# Autodesk Inventor assembly: Arm 2.0 Assembly
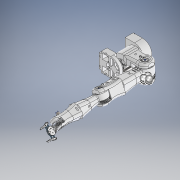
[picture p0: Inventor's stored thumbnail of the model, 180x180]
Saved by Autodesk Inventor 2017 SP1 (Build 210196100, 196)
## iProperties
Created: 2017-09-28
Part Number: Arm 2.0 Assembly
Document SubType Name: Assembly
Designer: Zach
Author: Zach
## Documents named in this file (49)
- C:\Users\Zach\Documents\GitHub\tr1\src\Body\Arm 2.0 Assembly\Arm 2.0 Assembly.iam
- C:\Users\Zach\Documents\GitHub\tr1\src\Body\Arm 2.0 Assembly\Steel Rod 8mm x 135mm.ipt
- C:\Users\Zach\Documents\GitHub\tr1\lib\22x8x8mm Bearing.ipt
- C:\Users\Zach\Documents\GitHub\tr1\src\Body\Arm 2.0 Assembly\AA004.ipt
- C:\Users\Zach\Documents\GitHub\tr1\lib\QS12MM250\QS12MM250.ipt
- C:\Users\Zach\Documents\GitHub\tr1\src\Body\Arm 2.0 Assembly\Steel Rod 8mm x 100mm.ipt
- C:\Users\Zach\Documents\GitHub\tr1\src\Body\Arm 2.0 Assembly\AA013.ipt
- C:\Users\Zach\Documents\GitHub\tr1\src\Body\Arm 2.0 Assembly\AA014.ipt
- C:\Users\Zach\Documents\GitHub\tr1\lib\12V DC Motor 378-1.ipt
- C:\Users\Zach\Documents\Inventor\Content Center Files\R2017\en-US\ISO 4017(1)\ISO 4017 - M5 x 20 - ISO.ipt
- C:\Users\Zach\Documents\GitHub\tr1\src\Body\Arm 2.0 Assembly\Steel Rod 8mm x 80mm.ipt
- C:\Users\Zach\Documents\GitHub\BCN3D-Moveo\Autodesk Inventor files\Gripper B Assembly.iam
- C:\Users\Zach\Documents\Inventor\Content Center Files\R2017\en-US\CNS 4320\CNS 4320 - M8 x 1 x 100.ipt
- C:\Users\Zach\Documents\GitHub\tr1\lib\AS 1110 - M8 x 150.ipt
- C:\Users\Zach\Documents\GitHub\tr1\lib\8mm Hub.ipt
- C:\Users\Zach\Documents\GitHub\tr1\src\Body\Arm 2.0 Assembly\Arm 2.0 Assembly\Design Accelerator\Spur Gears5.iam
- C:\Users\Zach\Documents\GitHub\tr1\lib\4mm mounting hub.ipt
- C:\Users\Zach\Documents\GitHub\tr1\lib\6201RS\6201RS.ipt
- C:\Users\Zach\Documents\GitHub\tr1\lib\U51105\U51105.ipt
- C:\Users\Zach\Documents\GitHub\tr1\src\Body\Arm 2.0 Assembly\AA031.ipt
- C:\Users\Zach\Documents\GitHub\tr1\src\Body\Arm 2.0 Assembly\AA034.ipt
- C:\Users\Zach\Documents\GitHub\tr1\src\Body\Arm 2.0 Assembly\Arm 2.0 Assembly\Design Accelerator\Spur Gears6.iam
- C:\Users\Zach\Documents\GitHub\tr1\src\Body\Arm 2.0 Assembly\AA008c.ipt
- C:\Users\Zach\Documents\GitHub\tr1\src\Body\Arm 2.0 Assembly\AA008d.ipt
- C:\Users\Zach\Documents\GitHub\tr1\src\Body\Arm 2.0 Assembly\AA035.ipt
- C:\Users\Zach\Documents\GitHub\tr1\src\Body\Arm 2.0 Assembly\Arm 2.0 Assembly\Design Accelerator\Spur Gears7.iam
- C:\Users\Zach\Documents\GitHub\tr1\src\Body\Arm 2.0 Assembly\AA036.ipt
- C:\Users\Zach\Documents\GitHub\tr1\src\Body\Arm 2.0 Assembly\AA037.ipt
- C:\Users\Zach\Documents\GitHub\tr1\src\Body\Arm 2.0 Assembly\AA016b.ipt
- C:\Users\Zach\Documents\GitHub\tr1\src\Body\Arm 2.0 Assembly\AA005b.ipt
- C:\Users\Zach\Documents\GitHub\tr1\src\Body\Arm 2.0 Assembly\AA006b.ipt
- C:\Users\Zach\Documents\GitHub\tr1\src\Body\Arm 2.0 Assembly\AA001c.ipt
- C:\Users\Zach\Documents\GitHub\tr1\lib\uxcell 12V 5RPM 8mm Worm Gear Motor\uxcell 12V 5RPM 8mm Worm Gear Motor.ipt
- C:\Users\Zach\Documents\GitHub\tr1\lib\Bourns ACE 128\Bourns ACE 128.ipt
- C:\Users\Zach\Documents\GitHub\tr1\src\Body\Arm 2.0 Assembly\Arm 2.0 Assembly\Design Accelerator\Spur Gears8.iam
- C:\Users\Zach\Documents\GitHub\tr1\src\Body\Arm 2.0 Assembly\Arm 2.0 Assembly\Design Accelerator\Spur Gears11.iam
- C:\Users\Zach\Documents\GitHub\tr1\src\Body\Arm 2.0 Assembly\Arm 2.0 Assembly\Design Accelerator\Spur Gears9.iam
- C:\Users\Zach\Documents\GitHub\tr1\src\Body\Arm 2.0 Assembly\AA010b.ipt
- C:\Users\Zach\Documents\GitHub\tr1\lib\uxcell 12V 6RPM 6mm Worm Gear Motor\uxcell 12V 6RPM 6mm Worm Gear Motor.ipt
- C:\Users\Zach\Documents\GitHub\tr1\src\Body\Arm 2.0 Assembly\Arm 2.0 Assembly\Design Accelerator\Spur Gears10.iam
- C:\Users\Zach\Documents\GitHub\tr1\src\Body\Arm 2.0 Assembly\Arm 2.0 Assembly\Design Accelerator\Spur Gears12.iam
- C:\Users\Zach\Documents\GitHub\tr1\src\Body\Arm 2.0 Assembly\AA041.ipt
- C:\Users\Zach\Documents\GitHub\tr1\src\Body\Arm 2.0 Assembly\AA042.ipt
- C:\Users\Zach\Documents\Inventor\Content Center Files\R2017\en-US\ISO 7045  H\ISO 7045 - M3 x 8 - 4.8 - H - ISO.ipt
- C:\Users\Zach\Documents\GitHub\tr1\src\Body\Arm 2.0 Assembly\AA043.ipt
- C:\Users\Zach\Documents\GitHub\tr1\src\Body\Arm 2.0 Assembly\AA044.ipt
- C:\Users\Zach\Documents\GitHub\tr1\src\Body\Arm 2.0 Assembly\AA045.ipt
- C:\Users\Zach\Documents\GitHub\tr1\src\Body\Arm 2.0 Assembly\Arm 2.0 Assembly\Design Accelerator\Spur Gears13.iam
- C:\Users\Zach\Documents\GitHub\tr1\src\Body\Arm 2.0 Assembly\Arm 2.0 Assembly\Design Accelerator\Spur Gears16.iam
## Components (84 placed, 39 different names)
1. AA001c:1 — Mate:554, Mate:555, Mate:556, Mate:557, Mate:560, Flush:18, Mate:562, Mate:563, Mate:564, Mate:565, Mate:566, Mate:567, Mate:568, Mate:569, Mate:570, Mate:571, Mate:572, Mate:573, Mate:574, Mate:576, Mate:578, Mate:581, Angle:1, Mate:592, Mate:602
2. AA004:1 — Mate:23, Mate:345, Mate:347, Mate:350, Mate:357, Mate:554, Mate:555, Mate:556, Mate:590, Mate:591
3. AA005b:1 — Mate:537, Mate:538, Mate:539, Mate:541, Mate:542, Mate:543
4. AA006b:1 — Mate:544, Mate:583, Mate:584, Angle:2, Mate:588, Mate:593, Mate:594, Mate:598, Mate:599, Mate:600, Mate:609
5. AA008c:1 — Mate:449, Mate:450, Mate:451, Mate:452, Mate:453, Mate:454, Mate:463, Mate:464, Mate:466, Mate:467, Mate:481, Mate:616, Mate:662, Mate:663
6. AA008d:1 — Mate:455, Mate:456, Mate:457, Mate:461, Mate:463, Mate:464, Mate:466, Mate:467, Mate:614, Angle:4, Mate:635, Mate:662, Mate:663, Mate:697, Mate:699
7. AA010b:1 — Mate:615, Mate:616, Mate:617, Mate:618, Mate:620, Mate:621, Mate:623, Mate:624, Mate:625, Mate:626, Mate:628, Mate:630, Mate:632, Mate:633, Mate:634, Mate:636, Mate:637, Angle:6, Mate:642, Flush:20, Mate:648, Mate:650
8. AA013:2 — Mate:142, Mate:143, Mate:144, Mate:145, Mate:146, Mate:147, Mate:563, Mate:564, Mate:565
9. AA014:2 — Mate:628, Mate:629, Mate:630
10. AA016b:1 — Mate:518, Mate:519, Mate:520, Mate:521, Mate:525, Mate:526, Mate:527, Mate:529, Mate:530, Mate:664, Mate:665, Mate:667, Mate:668, Mate:669, Angle:7, Mate:671, Mate:673, Mate:675, Mate:676, Mate:677
11. AA031:1 — Mate:366, Mate:367, Mate:523, Mate:524
12. AA034:1 — Mate:529, Mate:534, Mate:535, Mate:700, Mate:701, Mate:709
13. AA035:1 — Mate:477, Mate:479, Mate:481, Mate:557, Mate:601, Mate:652, Mate:653, Mate:697, Mate:699
14. AA036:1 — Mate:498, Mate:500, Mate:501, Mate:502, Mate:511, Mate:698
15. AA037:1 — Mate:501, Mate:502, Mate:514, Mate:515, Mate:516, Mate:517, Mate:518, Mate:519, Mate:520, Mate:530, Mate:664, Mate:665, Mate:698
16. AA041:1 — Mate:675, Mate:676, Mate:677, Mate:682, Mate:683, Mate:684, Mate:685
17. AA042:1 — Mate:678, Mate:679, Mate:686, Mate:687
18. AA043:1 — Mate:688, Mate:689, Angle:8
19. AA043:2 — Mate:693, Mate:694, Angle:10
20. AA044:1 — Mate:691, Mate:692, Angle:9
21. AA044:2 — Mate:695, Mate:696, Angle:11
22. AA045:2 — Mate:700, Mate:701, Mate:702, Mate:703, Mate:704, Mate:705, Mate:706, Mate:708, Flush:21, Mate:709, Mate:711, Mate:713, Mate:715, Mate:717, Mate:718, Angle:12, Mate:719, Mate:720, Mate:723, Mate:725
23. Gripper B Assembly:1 [sub-assembly]
24. 22x8x8mm Bearing:1 — Mate:433, Mate:560
25. 22x8x8mm Bearing:2 — Mate:437, Mate:562
26. 22x8x8mm Bearing:3 — Mate:57, Mate:620, Mate:626, Mate:645
27. 22x8x8mm Bearing:4 — Mate:621, Mate:629, Mate:642
28. 22x8x8mm Bearing:5 — Mate:186, Mate:708
29. 22x8x8mm Bearing:6 — Mate:187, Mate:719
30. 22x8x8mm Bearing:7 — Mate:264, Mate:526
31. 22x8x8mm Bearing:8 — Mate:527, Mate:528
32. 22x8x8mm Bearing:13 — Mate:451, Mate:452
33. 22x8x8mm Bearing:14 — Mate:449, Mate:450
34. QS12MM250:1 — Mate:23, Mate:344, Mate:346, Mate:348, Mate:354, Mate:537, Mate:544, Mate:585, Mate:593, Mate:594, Mate:597
35. Steel Rod 8mm x 135mm:1 — Mate:433, Mate:437, Mate:476, Mate:477, Flush:18, Mate:575, Mate:651
36. Steel Rod 8mm x 100mm:1 — Mate:57, Mate:491, Mate:498, Flush:20, Mate:644, Mate:649
37. Steel Rod 8mm x 80mm:1 — Mate:186, Mate:187, Mate:706, Flush:21, Mate:710, Mate:721, Mate:724
38. 12V DC Motor 378-1:3 — Mate:702, Mate:703, Mate:704, Mate:705, Mate:712, Mate:714
39. 12V DC Motor 378-1:4 — Mate:514, Mate:515, Mate:516, Mate:522
40. 12V DC Motor 378-1:6 — Mate:340, Mate:342, Mate:538, Mate:539, Mate:540, Mate:543
41. 12V DC Motor 378-1:7 — Mate:455, Mate:456, Mate:457, Mate:460, Mate:610
42. uxcell 12V 6RPM 6mm Worm Gear Motor:1 — Mate:632, Mate:633, Mate:634
43. uxcell 12V 5RPM 8mm Worm Gear Motor:1 — Mate:568, Mate:569, Mate:570, Mate:571, Mate:572
44. 6201RS:1 — Mate:346, Mate:347
45. 6201RS:2 — Mate:357, Mate:597
46. U51105:1 — Mate:348, Mate:349, Mate:542
47. U51105:2 — Mate:354, Mate:608, Mate:609
48. 8mm Hub:2 — Mate:368, Mate:531, Mate:534, Mate:535
49. 8mm Hub:3 — Mate:617, Mate:618, Mate:690
50. 8mm Hub:4 — Mate:580, Mate:581, Mate:582
51. 8mm Hub:5 — Mate:644, Mate:645, Mate:646
52. 8mm Hub:6 — Mate:651, Mate:652, Mate:653
53. 8mm Hub:7 — Mate:666, Mate:667, Mate:674
54. 8mm Hub:8 — Mate:720, Mate:721
55. 4mm mounting hub:1 — Mate:340, Mate:343, Mate:540, Mate:541
56. 4mm mounting hub:3 — Mate:366, Mate:367, Mate:517, Mate:522, Mate:523, Mate:524
57. 4mm mounting hub:5 — Mate:513, Mate:622, Mate:623
58. 4mm mounting hub:7 — Mate:460, Mate:461, Mate:611, Mate:613
59. 4mm mounting hub:8 — Mate:714, Mate:715, Mate:716
60. ISO 4017 M5 x 20:1 — Mate:146, Mate:147
61. ISO 4017 M5 x 20:2 — Mate:144, Mate:145
62. ISO 4017 M5 x 20:3 — Mate:142, Mate:143
63. CNS 4320 M8 x 100:1 — Mate:264, Mate:368, Mate:521, Mate:525, Mate:528, Mate:531, Mate:666, Mate:670
64. AS 1110 - Metric M8 x 80:2 — Mate:453, Mate:454, Angle:5, Mate:615, Mate:690
65. ISO 7045 H M3 x 8 - 4.8 - H:1 — Mate:680, Mate:681
66. ISO 7045 H M3 x 8 - 4.8 - H:2 — Mate:682, Mate:685
67. ISO 7045 H M3 x 8 - 4.8 - H:3 — Mate:683, Mate:684
68. ISO 7045 H M3 x 8 - 4.8 - H:4 — Mate:686, Mate:687
69. Bourns ACE 128:1 — Mate:573, Mate:574, Mate:577, Angle:1, Mate:693, Mate:694
70. Bourns ACE 128:2 — Mate:583, Mate:584, Angle:2, Mate:587, Mate:695, Mate:696
71. Bourns ACE 128:3 — Mate:612, Mate:614, Angle:4, Mate:635, Mate:691, Mate:692
72. Bourns ACE 128:4 — Mate:636, Mate:637, Angle:6, Mate:647, Mate:688, Mate:689
73. Bourns ACE 128:5 — Mate:668, Mate:669, Angle:7, Mate:672, Mate:678, Mate:679
74. Bourns ACE 128:6 — Mate:717, Mate:718, Angle:12, Mate:722
75. Spur Gears:5 [sub-assembly] — Mate:342, Mate:343, Mate:344, Mate:345, Mate:349, Mate:350
76. Spur Gears:6 [sub-assembly] — Mate:476, Mate:479, Mate:566, Mate:567, Mate:601, Mate:602
77. Spur Gears:7 [sub-assembly] — Mate:491, Mate:500, Mate:511, Mate:513, Mate:622, Mate:624, Mate:625
78. Spur Gears:8 [sub-assembly] — Mate:575, Mate:576, Mate:577, Mate:578, Mate:580, Mate:582, Angle:10
79. Spur Gears:9 [sub-assembly] — Mate:585, Mate:587, Mate:588, Mate:590, Mate:591, Mate:592, Mate:608, Angle:11
80. Spur Gears:10 [sub-assembly] — Mate:610, Mate:611, Mate:612, Mate:613, Angle:5, Angle:9
81. Spur Gears:11 [sub-assembly] — Mate:646, Mate:647, Mate:648, Mate:649, Mate:650, Angle:8
82. Spur Gears:12 [sub-assembly] — Mate:670, Mate:671, Mate:672, Mate:673, Mate:674, Mate:680, Mate:681
83. Spur Gears:13 [sub-assembly] — Mate:710, Mate:711, Mate:712, Mate:713, Mate:716
84. Spur Gears:14 [sub-assembly] — Mate:722, Mate:723, Mate:724, Mate:725
## Relationships (238: Mate 224, Angle 11, Flush 3)
- Mate:23: AA004:1 ↔ QS12MM250:1
- Mate:57: 22x8x8mm Bearing:3 ↔ Steel Rod 8mm x 100mm:1
- Mate:142: AA013:2 ↔ ISO 4017 M5 x 20:3
- Mate:143: AA013:2 ↔ ISO 4017 M5 x 20:3
- Mate:144: AA013:2 ↔ ISO 4017 M5 x 20:2
- Mate:145: AA013:2 ↔ ISO 4017 M5 x 20:2
- Mate:146: AA013:2 ↔ ISO 4017 M5 x 20:1
- Mate:147: AA013:2 ↔ ISO 4017 M5 x 20:1
- Mate:186: 22x8x8mm Bearing:5 ↔ Steel Rod 8mm x 80mm:1
- Mate:187: 22x8x8mm Bearing:6 ↔ Steel Rod 8mm x 80mm:1
- Mate:264: 22x8x8mm Bearing:7 ↔ CNS 4320 M8 x 100:1
- Mate:340: 12V DC Motor 378-1:6 ↔ 4mm mounting hub:1
- Mate:342: 12V DC Motor 378-1:6 ↔ Spur Gears:5
- Mate:343: 4mm mounting hub:1 ↔ Spur Gears:5
- Mate:344: QS12MM250:1 ↔ Spur Gears:5
- Mate:345: AA004:1 ↔ Spur Gears:5
- Mate:346: QS12MM250:1 ↔ 6201RS:1
- Mate:347: AA004:1 ↔ 6201RS:1
- Mate:348: QS12MM250:1 ↔ U51105:1
- Mate:349: U51105:1 ↔ Spur Gears:5
- Mate:350: AA004:1 ↔ Spur Gears:5
- Mate:354: QS12MM250:1 ↔ U51105:2
- Mate:357: AA004:1 ↔ 6201RS:2
- Mate:366: AA031:1 ↔ 4mm mounting hub:3
- Mate:367: AA031:1 ↔ 4mm mounting hub:3
- Mate:368: 8mm Hub:2 ↔ CNS 4320 M8 x 100:1
- Mate:433: 22x8x8mm Bearing:1 ↔ Steel Rod 8mm x 135mm:1
- Mate:437: 22x8x8mm Bearing:2 ↔ Steel Rod 8mm x 135mm:1
- Mate:449: AA008c:1 ↔ 22x8x8mm Bearing:14
- Mate:450: AA008c:1 ↔ 22x8x8mm Bearing:14
- Mate:451: AA008c:1 ↔ 22x8x8mm Bearing:13
- Mate:452: AA008c:1 ↔ 22x8x8mm Bearing:13
- Mate:453: AA008c:1 ↔ AS 1110 - Metric M8 x 80:2
- Mate:454: AA008c:1 ↔ AS 1110 - Metric M8 x 80:2
- Mate:455: AA008d:1 ↔ 12V DC Motor 378-1:7
- Mate:456: AA008d:1 ↔ 12V DC Motor 378-1:7
- Mate:457: AA008d:1 ↔ 12V DC Motor 378-1:7
- Mate:460: 12V DC Motor 378-1:7 ↔ 4mm mounting hub:7
- Mate:461: AA008d:1 ↔ 4mm mounting hub:7
- Mate:463: AA008c:1 ↔ AA008d:1
- Mate:464: AA008c:1 ↔ AA008d:1
- Mate:466: AA008c:1 ↔ AA008d:1
- Mate:467: AA008c:1 ↔ AA008d:1
- Mate:476: Steel Rod 8mm x 135mm:1 ↔ Spur Gears:6
- Mate:477: AA035:1 ↔ Steel Rod 8mm x 135mm:1
- Mate:479: AA035:1 ↔ Spur Gears:6
- Mate:481: AA008c:1 ↔ AA035:1
- Mate:491: Steel Rod 8mm x 100mm:1 ↔ Spur Gears:7
- Mate:498: AA036:1 ↔ Steel Rod 8mm x 100mm:1
- Mate:500: AA036:1 ↔ Spur Gears:7
- Mate:501: AA036:1 ↔ AA037:1
- Mate:502: AA036:1 ↔ AA037:1
- Mate:511: AA036:1 ↔ Spur Gears:7
- Mate:513: 4mm mounting hub:5 ↔ Spur Gears:7
- Mate:514: AA037:1 ↔ 12V DC Motor 378-1:4
- Mate:515: AA037:1 ↔ 12V DC Motor 378-1:4
- Mate:516: AA037:1 ↔ 12V DC Motor 378-1:4
- Mate:517: AA037:1 ↔ 4mm mounting hub:3
- Mate:518: AA016b:1 ↔ AA037:1
- Mate:519: AA016b:1 ↔ AA037:1
- Mate:520: AA016b:1 ↔ AA037:1
- Mate:521: AA016b:1 ↔ CNS 4320 M8 x 100:1
- Mate:522: 12V DC Motor 378-1:4 ↔ 4mm mounting hub:3
- Mate:523: AA031:1 ↔ 4mm mounting hub:3
- Mate:524: AA031:1 ↔ 4mm mounting hub:3
- Mate:525: AA016b:1 ↔ CNS 4320 M8 x 100:1
- Mate:526 (0.5 mm): AA016b:1 ↔ 22x8x8mm Bearing:7
- Mate:527 (0.5 mm): AA016b:1 ↔ 22x8x8mm Bearing:8
- Mate:528: 22x8x8mm Bearing:8 ↔ CNS 4320 M8 x 100:1
- Mate:529: AA016b:1 ↔ AA034:1
- Mate:530: AA016b:1 ↔ AA037:1
- Mate:531: 8mm Hub:2 ↔ CNS 4320 M8 x 100:1
- Mate:534: AA034:1 ↔ 8mm Hub:2
- Mate:535: AA034:1 ↔ 8mm Hub:2
- Mate:537: AA005b:1 ↔ QS12MM250:1
- Mate:538: AA005b:1 ↔ 12V DC Motor 378-1:6
- Mate:539: AA005b:1 ↔ 12V DC Motor 378-1:6
- Mate:540: 12V DC Motor 378-1:6 ↔ 4mm mounting hub:1
- Mate:541: AA005b:1 ↔ 4mm mounting hub:1
- Mate:542: AA005b:1 ↔ U51105:1
- Mate:543: AA005b:1 ↔ 12V DC Motor 378-1:6
- Mate:544: AA006b:1 ↔ QS12MM250:1
- Mate:554: AA001c:1 ↔ AA004:1
- Mate:555: AA001c:1 ↔ AA004:1
- Mate:556: AA001c:1 ↔ AA004:1
- Mate:557: AA001c:1 ↔ AA035:1
- Mate:560: AA001c:1 ↔ 22x8x8mm Bearing:1
- Flush:18: AA001c:1 ↔ Steel Rod 8mm x 135mm:1
- Mate:562: AA001c:1 ↔ 22x8x8mm Bearing:2
- Mate:563: AA001c:1 ↔ AA013:2
- Mate:564: AA001c:1 ↔ AA013:2
- Mate:565: AA001c:1 ↔ AA013:2
- Mate:566: AA001c:1 ↔ Spur Gears:6
- Mate:567 (1 mm): AA001c:1 ↔ Spur Gears:6
- Mate:568: AA001c:1 ↔ uxcell 12V 5RPM 8mm Worm Gear Motor:1
- Mate:569: AA001c:1 ↔ uxcell 12V 5RPM 8mm Worm Gear Motor:1
- Mate:570: AA001c:1 ↔ uxcell 12V 5RPM 8mm Worm Gear Motor:1
- Mate:571: AA001c:1 ↔ uxcell 12V 5RPM 8mm Worm Gear Motor:1
- Mate:572: AA001c:1 ↔ uxcell 12V 5RPM 8mm Worm Gear Motor:1
- Mate:573: AA001c:1 ↔ Bourns ACE 128:1
- Mate:574: AA001c:1 ↔ Bourns ACE 128:1
- Mate:575: Steel Rod 8mm x 135mm:1 ↔ Spur Gears:8
- Mate:576: AA001c:1 ↔ Spur Gears:8
- Mate:577: Bourns ACE 128:1 ↔ Spur Gears:8
- Mate:578: AA001c:1 ↔ Spur Gears:8
- Mate:580: 8mm Hub:4 ↔ Spur Gears:8
- Mate:581: AA001c:1 ↔ 8mm Hub:4
- Mate:582: 8mm Hub:4 ↔ Spur Gears:8
- Angle:1 (0 deg): AA001c:1 ↔ Bourns ACE 128:1
- Mate:583: AA006b:1 ↔ Bourns ACE 128:2
- Mate:584: AA006b:1 ↔ Bourns ACE 128:2
- Angle:2 (0 deg): AA006b:1 ↔ Bourns ACE 128:2
- Mate:585: QS12MM250:1 ↔ Spur Gears:9
- Mate:587: Bourns ACE 128:2 ↔ Spur Gears:9
- Mate:588: AA006b:1 ↔ Spur Gears:9
- Mate:590: AA004:1 ↔ Spur Gears:9
- Mate:591: AA004:1 ↔ Spur Gears:9
- Mate:592: AA001c:1 ↔ Spur Gears:9
- Mate:593: AA006b:1 ↔ QS12MM250:1
- Mate:594: AA006b:1 ↔ QS12MM250:1
- Mate:597: QS12MM250:1 ↔ 6201RS:2
- Mate:598: AA006b:1
- Mate:599: AA006b:1
- Mate:600: AA006b:1
- Mate:601: AA035:1 ↔ Spur Gears:6
- Mate:602 (2.5 mm): AA001c:1 ↔ Spur Gears:6
- Mate:608: U51105:2 ↔ Spur Gears:9
- Mate:609: AA006b:1 ↔ U51105:2
- Mate:610: 12V DC Motor 378-1:7 ↔ Spur Gears:10
- Mate:611: 4mm mounting hub:7 ↔ Spur Gears:10
- Mate:612: Bourns ACE 128:3 ↔ Spur Gears:10
- Mate:613: 4mm mounting hub:7 ↔ Spur Gears:10
- Mate:614: AA008d:1 ↔ Bourns ACE 128:3
- Angle:4 (0 deg): AA008d:1 ↔ Bourns ACE 128:3
- Angle:5 (0 deg): AS 1110 - Metric M8 x 80:2 ↔ Spur Gears:10
- Mate:615: AA010b:1 ↔ AS 1110 - Metric M8 x 80:2
- Mate:616: AA008c:1 ↔ AA010b:1
- Mate:617: AA010b:1 ↔ 8mm Hub:3
- Mate:618: AA010b:1 ↔ 8mm Hub:3
- Mate:620: AA010b:1 ↔ 22x8x8mm Bearing:3
- Mate:621: AA010b:1 ↔ 22x8x8mm Bearing:4
- Mate:622: 4mm mounting hub:5 ↔ Spur Gears:7
- Mate:623: AA010b:1 ↔ 4mm mounting hub:5
- Mate:624: AA010b:1 ↔ Spur Gears:7
- Mate:625: AA010b:1 ↔ Spur Gears:7
- Flush:20 (0.5 mm): AA010b:1 ↔ Steel Rod 8mm x 100mm:1
- Mate:626: AA010b:1 ↔ 22x8x8mm Bearing:3
- Mate:628: AA010b:1 ↔ AA014:2
- Mate:629: AA014:2 ↔ 22x8x8mm Bearing:4
- Mate:630: AA010b:1 ↔ AA014:2
- Mate:632: AA010b:1 ↔ uxcell 12V 6RPM 6mm Worm Gear Motor:1
- Mate:633: AA010b:1 ↔ uxcell 12V 6RPM 6mm Worm Gear Motor:1
- Mate:634: AA010b:1 ↔ uxcell 12V 6RPM 6mm Worm Gear Motor:1
- Mate:635: AA008d:1 ↔ Bourns ACE 128:3
- Mate:636: AA010b:1 ↔ Bourns ACE 128:4
- Mate:637: AA010b:1 ↔ Bourns ACE 128:4
- Angle:6 (0 deg): AA010b:1 ↔ Bourns ACE 128:4
- Mate:642: AA010b:1 ↔ 22x8x8mm Bearing:4
- Mate:644: Steel Rod 8mm x 100mm:1 ↔ 8mm Hub:5
- Mate:645: 22x8x8mm Bearing:3 ↔ 8mm Hub:5
- Mate:646: 8mm Hub:5 ↔ Spur Gears:11
- Mate:647: Bourns ACE 128:4 ↔ Spur Gears:11
- Mate:648: AA010b:1 ↔ Spur Gears:11
- Mate:649: Steel Rod 8mm x 100mm:1 ↔ Spur Gears:11
- Mate:650: AA010b:1 ↔ Spur Gears:11
- Mate:651: Steel Rod 8mm x 135mm:1 ↔ 8mm Hub:6
- Mate:652: AA035:1 ↔ 8mm Hub:6
- Mate:653: AA035:1 ↔ 8mm Hub:6
- Mate:662: AA008c:1 ↔ AA008d:1
- Mate:663: AA008c:1 ↔ AA008d:1
- Mate:664: AA016b:1 ↔ AA037:1
- Mate:665: AA016b:1 ↔ AA037:1
- Mate:666: 8mm Hub:7 ↔ CNS 4320 M8 x 100:1
- Mate:667: AA016b:1 ↔ 8mm Hub:7
- Mate:668: AA016b:1 ↔ Bourns ACE 128:5
- Mate:669: AA016b:1 ↔ Bourns ACE 128:5
- Angle:7 (0 deg): AA016b:1 ↔ Bourns ACE 128:5
- Mate:670: CNS 4320 M8 x 100:1 ↔ Spur Gears:12
- Mate:671: AA016b:1 ↔ Spur Gears:12
- Mate:672: Bourns ACE 128:5 ↔ Spur Gears:12
- Mate:673: AA016b:1 ↔ Spur Gears:12
- Mate:674: 8mm Hub:7 ↔ Spur Gears:12
- Mate:675: AA016b:1 ↔ AA041:1
- Mate:676: AA016b:1 ↔ AA041:1
- Mate:677: AA016b:1 ↔ AA041:1
- Mate:678: AA042:1 ↔ Bourns ACE 128:5
- Mate:679: AA042:1 ↔ Bourns ACE 128:5
- Mate:680: ISO 7045 H M3 x 8 - 4.8 - H:1 ↔ Spur Gears:12
- Mate:681: ISO 7045 H M3 x 8 - 4.8 - H:1 ↔ Spur Gears:12
- Mate:682: AA041:1 ↔ ISO 7045 H M3 x 8 - 4.8 - H:2
- Mate:683: AA041:1 ↔ ISO 7045 H M3 x 8 - 4.8 - H:3
- Mate:684: AA041:1 ↔ ISO 7045 H M3 x 8 - 4.8 - H:3
- Mate:685: AA041:1 ↔ ISO 7045 H M3 x 8 - 4.8 - H:2
- Mate:686: AA042:1 ↔ ISO 7045 H M3 x 8 - 4.8 - H:4
- Mate:687: AA042:1 ↔ ISO 7045 H M3 x 8 - 4.8 - H:4
- Mate:688: AA043:1 ↔ Bourns ACE 128:4
- Mate:689: AA043:1 ↔ Bourns ACE 128:4
- Angle:8 (0 deg): AA043:1 ↔ Spur Gears:11
- Mate:690: 8mm Hub:3 ↔ AS 1110 - Metric M8 x 80:2
- Mate:691: AA044:1 ↔ Bourns ACE 128:3
- Mate:692: AA044:1 ↔ Bourns ACE 128:3
- Angle:9 (0 deg): AA044:1 ↔ Spur Gears:10
- Mate:693: AA043:2 ↔ Bourns ACE 128:1
- Mate:694: AA043:2 ↔ Bourns ACE 128:1
- Angle:10 (0 deg): AA043:2 ↔ Spur Gears:8
- Mate:695: AA044:2 ↔ Bourns ACE 128:2
- Mate:696: AA044:2 ↔ Bourns ACE 128:2
- Angle:11 (0 deg): AA044:2 ↔ Spur Gears:9
- Mate:697: AA008d:1 ↔ AA035:1
- Mate:698: AA036:1 ↔ AA037:1
- Mate:699: AA008d:1 ↔ AA035:1
- Mate:700: AA034:1 ↔ AA045:2
- Mate:701: AA034:1 ↔ AA045:2
- Mate:702: AA045:2 ↔ 12V DC Motor 378-1:3
- Mate:703: AA045:2 ↔ 12V DC Motor 378-1:3
- Mate:704: AA045:2 ↔ 12V DC Motor 378-1:3
- Mate:705: AA045:2 ↔ 12V DC Motor 378-1:3
- Mate:706: AA045:2 ↔ Steel Rod 8mm x 80mm:1
- Mate:708: AA045:2 ↔ 22x8x8mm Bearing:5
- Flush:21: AA045:2 ↔ Steel Rod 8mm x 80mm:1
- Mate:709: AA034:1 ↔ AA045:2
- Mate:710: Steel Rod 8mm x 80mm:1 ↔ Spur Gears:13
- Mate:711: AA045:2 ↔ Spur Gears:13
- Mate:712: 12V DC Motor 378-1:3 ↔ Spur Gears:13
- Mate:713: AA045:2 ↔ Spur Gears:13
- Mate:714: 12V DC Motor 378-1:3 ↔ 4mm mounting hub:8
- Mate:715: AA045:2 ↔ 4mm mounting hub:8
- Mate:716: 4mm mounting hub:8 ↔ Spur Gears:13
- Mate:717: AA045:2 ↔ Bourns ACE 128:6
- Mate:718: AA045:2 ↔ Bourns ACE 128:6
- Angle:12 (0 deg): AA045:2 ↔ Bourns ACE 128:6
- Mate:719: AA045:2 ↔ 22x8x8mm Bearing:6
- Mate:720: AA045:2 ↔ 8mm Hub:8
- Mate:721: Steel Rod 8mm x 80mm:1 ↔ 8mm Hub:8
- Mate:722: Bourns ACE 128:6 ↔ Spur Gears:14
- Mate:723: AA045:2 ↔ Spur Gears:14
- Mate:724: Steel Rod 8mm x 80mm:1 ↔ Spur Gears:14
- Mate:725: AA045:2 ↔ Spur Gears:14
